# Autodesk Inventor assembly: 4 Omni AS, Square_MIR1
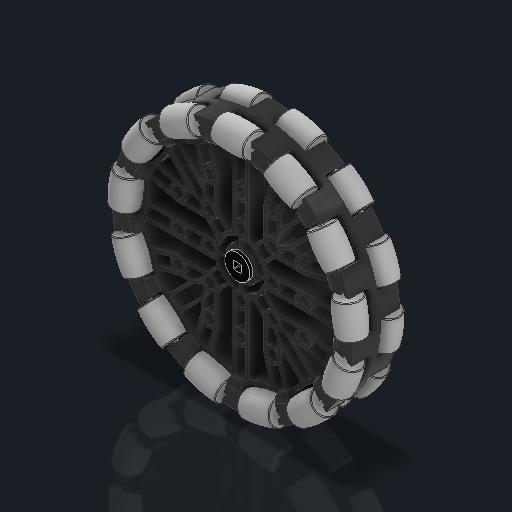
[picture p0: Inventor's stored thumbnail of the model, 512x512]
Saved by Autodesk Inventor 2023.2 (Build 272271030, 271C)
## iProperties
Created: 2022-08-02
Part Number: 4 Omni AS, Square_MIR1
Document SubType Name: Assembly
Designer: Michael
Author: ylu12
## Documents named in this file (3)
- C:\Users\black\OneDrive\Pictures\Documents\VEX CAD\VEX-CAD-Inventor-1.4.0\Motion\Wheels\Omni Wheel\4 Omni AS, Square_MIR1.iam
- C:\Users\black\OneDrive\Pictures\Documents\VEX CAD\VEX-CAD-Inventor-1.4.0\Motion\Wheels\Reference Files\4 Omni Antistatic_MIR1.ipt
- C:\Users\black\OneDrive\Pictures\Documents\VEX CAD\VEX-CAD-Inventor-1.4.0\Motion\Insert Square_MIR1.ipt
## Components (3 placed, 2 different names)
1. 4 Omni Antistatic_MIR1:1 — Mate:14, Mate:13, Flush:7
2. Insert Square_MIR1:1 — Flush:11, Flush:10, Mate:17
3. Insert Square_MIR1:2 — Angle:1, Mate:18, Flush:11, Flush:10, Flush:9
## Relationships (9: Mate 4, Flush 4, Angle 1)
- Mate:14: 4 Omni Antistatic_MIR1:1
- Mate:13: 4 Omni Antistatic_MIR1:1
- Flush:7: 4 Omni Antistatic_MIR1:1
- Angle:1 (0 deg): Insert Square_MIR1:2
- Mate:18: Insert Square_MIR1:2
- Flush:11: Insert Square_MIR1:1 ↔ Insert Square_MIR1:2
- Flush:10: Insert Square_MIR1:1 ↔ Insert Square_MIR1:2
- Flush:9 [Mate] (6.35 mm): Insert Square_MIR1:2
- Mate:17 [Flush] (6.35 mm): Insert Square_MIR1:1
